# Autodesk Inventor assembly: roller-hand-v2-P
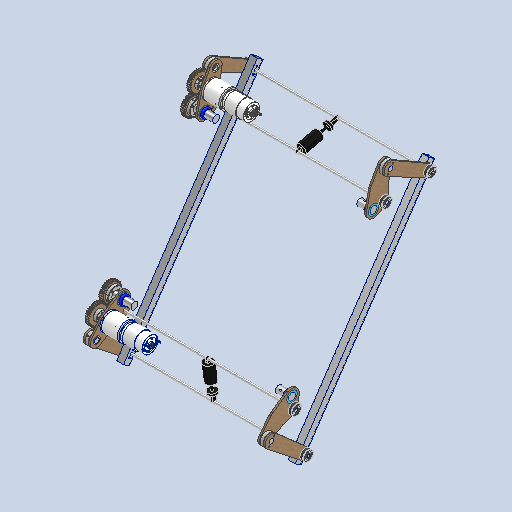
[picture p0: Inventor's stored thumbnail of the model, 512x512]
Saved by Autodesk Inventor 2025.1 (Build 291241000, 241)
## iProperties
Created: 2024-10-06
Part Number: roller-hand-v2-P
Document SubType Name: Assembly
Designer: haruy
Author: haruy
## Documents named in this file (38)
- C:\Users\haruy\Documents\ロボコン\NHK2025\cad\nagahisa\hand\roller\roller-hand-v2-P.iam
- C:\Users\haruy\Documents\ロボコン\NHK2025\cad\nagahisa\hand\roller\roller-hand-v1-MDF-m385-m.ipt
- C:\Users\haruy\Documents\ロボコン\NHK2025\cad\nagahisa\hand\roller\roller-hand-v2-MDF-link-1.ipt
- C:\Users\haruy\Documents\ロボコン\NHK2025\cad\nagahisa\hand\roller\roller-hand-v2-MDF-m385-r.ipt
- C:\Users\haruy\Documents\ロボコン\NHK2025\cad\nagahisa\hand\roller\SCSWJ8-6_b.ipt
- C:\Users\haruy\Documents\ロボコン\NHK2025\cad\000_parts\ベアリング\8\bear_f8_12_sa.ipt
- C:\Users\haruy\Documents\ロボコン\NHK2025\cad\000_parts\モーター\Geared_RS-385.iam
- C:\Users\haruy\Documents\ロボコン\NHK2025\cad\nagahisa\hand\roller\SCSWJ6-6_b.ipt
- C:\Users\haruy\Documents\ロボコン\NHK2025\cad\000_parts\ベアリング\12\TH22_bearing_12_18_19.5_sn.ipt
- C:\Users\haruy\Documents\ロボコン\NHK2025\cad\nagahisa\hand\roller\roller-hand-v2-Shaft-link1.ipt
- C:\Users\haruy\Documents\ロボコン\NHK2025\cad\nagahisa\hand\roller\roller-hand-v2-Shaft-link2.ipt
- C:\Users\haruy\Documents\ロボコン\NHK2025\cad\nagahisa\hand\roller\roller-hand-v2-Shaft-m.ipt
- C:\Users\haruy\Documents\ロボコン\NHK2025\cad\nagahisa\hand\roller\SCSWJ12-6_b.ipt
- C:\Users\haruy\Documents\ロボコン\NHK2025\cad\000_parts\サスペンション\black-suspension.iam
- C:\Users\haruy\Documents\ロボコン\NHK2025\cad\nagahisa\hand\roller\roller-hand-v2-Shaft-link3.ipt
- C:\Users\haruy\Documents\ロボコン\NHK2025\cad\nagahisa\hand\roller\roller-hand-v2-Shaft-m-r.ipt
- C:\Users\haruy\Documents\ロボコン\NHK2025\cad\nagahisa\hand\roller\roller-hand-v2-ASP-1.ipt
- C:\Users\haruy\Documents\ロボコン\NHK2025\cad\nagahisa\hand\roller\SCSWJ4-6_b.ipt
- C:\Users\haruy\Documents\ロボコン\NHK2025\cad\nagahisa\hand\roller\roller-hand-v2-P\デザイン アクセラレータ\平歯車1.iam
- C:\Users\haruy\Documents\ロボコン\NHK2025\cad\nagahisa\hand\roller\roller-hand-v2-3DP-shaft-spesa.ipt
- C:\Users\haruy\Documents\ロボコン\NHK2025\cad\nagahisa\hand\roller\roller-hand-v1-MDF-m385-m_MIR.ipt
- C:\Users\haruy\Documents\ロボコン\NHK2025\cad\nagahisa\hand\roller\roller-hand-v2-MDF-link-1_MIR.ipt
- C:\Users\haruy\Documents\ロボコン\NHK2025\cad\nagahisa\hand\roller\roller-hand-v2-MDF-m385-r_MIR.ipt
- C:\Users\haruy\Documents\ロボコン\NHK2025\cad\nagahisa\hand\roller\SCSWJ8-6_b_MIR.ipt
- C:\Users\haruy\Documents\ロボコン\NHK2025\cad\000_parts\モーター\Geared_RS-385_MIR.iam
- C:\Users\haruy\Documents\ロボコン\NHK2025\cad\nagahisa\hand\roller\SCSWJ6-6_b_MIR.ipt
- C:\Users\haruy\Documents\ロボコン\NHK2025\cad\000_parts\ベアリング\12\TH22_bearing_12_18_19.5_sn_MIR.ipt
- C:\Users\haruy\Documents\ロボコン\NHK2025\cad\nagahisa\hand\roller\roller-hand-v2-Shaft-link1_MIR.ipt
- C:\Users\haruy\Documents\ロボコン\NHK2025\cad\000_parts\ベアリング\8\bear_f8_12_sa_MIR.ipt
- C:\Users\haruy\Documents\ロボコン\NHK2025\cad\nagahisa\hand\roller\roller-hand-v2-Shaft-link2_MIR.ipt
- C:\Users\haruy\Documents\ロボコン\NHK2025\cad\nagahisa\hand\roller\roller-hand-v2-Shaft-m_MIR.ipt
- C:\Users\haruy\Documents\ロボコン\NHK2025\cad\nagahisa\hand\roller\SCSWJ12-6_b_MIR.ipt
- C:\Users\haruy\Documents\ロボコン\NHK2025\cad\000_parts\サスペンション\black-suspension_MIR.iam
- C:\Users\haruy\Documents\ロボコン\NHK2025\cad\nagahisa\hand\roller\roller-hand-v2-Shaft-link3_MIR.ipt
- C:\Users\haruy\Documents\ロボコン\NHK2025\cad\nagahisa\hand\roller\roller-hand-v2-Shaft-m-r_MIR.ipt
- C:\Users\haruy\Documents\ロボコン\NHK2025\cad\nagahisa\hand\roller\SCSWJ4-6_b_MIR.ipt
- C:\Users\haruy\Documents\ロボコン\NHK2025\cad\nagahisa\hand\roller\roller-hand-v2-P\デザイン アクセラレータ\平歯車1_MIR.iam
- C:\Users\haruy\Documents\ロボコン\NHK2025\cad\nagahisa\hand\roller\roller-hand-v2-3DP-shaft-spesa_MIR.ipt
## Components (55 placed, 37 different names)
1. roller-hand-v1-MDF-m385-m:1 — 挿入:4, 挿入:6, 挿入:8, 挿入:16, 挿入:21, 挿入:35
2. roller-hand-v2-MDF-link-1:1 — 挿入:7, 挿入:10, 挿入:22, 挿入:23, 挿入:27, 挿入:28, 挿入:34
3. roller-hand-v2-MDF-m385-r:1 — 挿入:12, 挿入:18, 挿入:25, 挿入:37
4. SCSWJ8-6_b:1 — 挿入:7, 挿入:9
5. bear_f8_12_sa:1 — 挿入:8, 挿入:9
6. Geared_RS-385:1 [sub-assembly] — 挿入:4, 挿入:5, メイト:1
7. SCSWJ6-6_b:1 — 挿入:5, メイト:2
8. TH22_bearing_12_18_19.5_sn:1 — 挿入:6, 挿入:19, 挿入:38, 挿入:39
9. roller-hand-v2-Shaft-link1:1 — 挿入:10, 挿入:29
10. TH22_bearing_12_18_19.5_sn:2 — 挿入:25, 挿入:26, 挿入:40
11. bear_f8_12_sa:2 — 挿入:12, 挿入:13
12. SCSWJ8-6_b:2 — 挿入:13, 挿入:31
13. roller-hand-v2-MDF-link-1:2 — 挿入:29, 挿入:30, 挿入:31, 挿入:32, 挿入:33, 挿入:36
14. roller-hand-v2-Shaft-link2:1 — 挿入:16, 挿入:18
15. roller-hand-v2-Shaft-m:1 — 挿入:19, メイト:3
16. SCSWJ12-6_b:1 — 挿入:38
17. black-suspension:1 [sub-assembly] — 挿入:21, 挿入:22
18. roller-hand-v2-Shaft-link3:1 — 挿入:23
19. roller-hand-v2-Shaft-link3:2 — 挿入:30
20. roller-hand-v2-Shaft-m-r:1 — 挿入:26
21. roller-hand-v2-ASP-1:1 — 挿入:27, 挿入:28, フラッシュ:1
22. roller-hand-v2-ASP-1:2 — 挿入:32, 挿入:33, 挿入:64, 挿入:65
23. SCSWJ4-6_b:1 — 挿入:35
24. SCSWJ4-6_b:2 — 挿入:34
25. SCSWJ4-6_b:3 — 挿入:36
26. SCSWJ4-6_b:4 — 挿入:37
27. 平歯車:1 [sub-assembly] — メイト:1, メイト:2, メイト:3
28. roller-hand-v2-3DP-shaft-spesa:1 — 挿入:39
29. roller-hand-v2-3DP-shaft-spesa:2 — 挿入:40
30. roller-hand-v1-MDF-m385-m_MIR:1 — 挿入:42, 挿入:44, 挿入:52, 挿入:56, 挿入:59, 挿入:66
31. roller-hand-v2-MDF-link-1_MIR:1 — 挿入:41, 挿入:45, 挿入:55, 挿入:60
32. roller-hand-v2-MDF-m385-r_MIR:1 — 挿入:46, 挿入:47, 挿入:51, 挿入:61
33. SCSWJ8-6_b_MIR:1 — 挿入:41, 挿入:67
34. Geared_RS-385_MIR:1 [sub-assembly] — 挿入:42, 挿入:43, メイト:6
35. SCSWJ6-6_b_MIR:1 — 挿入:43, メイト:5
36. TH22_bearing_12_18_19.5_sn_MIR:1 — 挿入:44, 挿入:53, 挿入:54, 挿入:62
37. roller-hand-v2-Shaft-link1_MIR:1 — 挿入:45, 挿入:50
38. TH22_bearing_12_18_19.5_sn_MIR:2 — 挿入:46, 挿入:58, 挿入:63
39. bear_f8_12_sa_MIR:1 — 挿入:47, 挿入:48
40. SCSWJ8-6_b_MIR:2 — 挿入:48, 挿入:49
41. roller-hand-v2-MDF-link-1_MIR:2 — 挿入:49, 挿入:50, 挿入:57, 挿入:64, 挿入:65, 挿入:68
42. roller-hand-v2-Shaft-link2_MIR:1 — 挿入:51, 挿入:52
43. roller-hand-v2-Shaft-m_MIR:1 — 挿入:53, メイト:4
44. SCSWJ12-6_b_MIR:1 — 挿入:54
45. black-suspension_MIR:1 [sub-assembly] — 挿入:55, 挿入:56
46. roller-hand-v2-Shaft-link3_MIR:1 — 挿入:57
47. roller-hand-v2-Shaft-m-r_MIR:1 — 挿入:58
48. SCSWJ4-6_b_MIR:1 — 挿入:59
49. SCSWJ4-6_b_MIR:2 — 挿入:60
50. SCSWJ4-6_b_MIR:3 — 挿入:61
51. 平歯車1_MIR:1 [sub-assembly] — メイト:4, メイト:5, メイト:6
52. roller-hand-v2-3DP-shaft-spesa_MIR:1 — 挿入:62
53. roller-hand-v2-3DP-shaft-spesa_MIR:2 — 挿入:63
54. bear_f8_12_sa:3 — 挿入:66, 挿入:67
55. SCSWJ4-6_b:5 — 挿入:68
## Relationships (66: Insert 59, Mate 6, Flush 1)
- 挿入:4 [Insert]: roller-hand-v1-MDF-m385-m:1 ↔ Geared_RS-385:1
- 挿入:5 [Insert] (8.8 mm): Geared_RS-385:1 ↔ SCSWJ6-6_b:1
- 挿入:6 [Insert]: roller-hand-v1-MDF-m385-m:1 ↔ TH22_bearing_12_18_19.5_sn:1
- 挿入:7 [Insert]: roller-hand-v2-MDF-link-1:1 ↔ SCSWJ8-6_b:1
- 挿入:8 [Insert]: roller-hand-v1-MDF-m385-m:1 ↔ bear_f8_12_sa:1
- 挿入:9 [Insert]: SCSWJ8-6_b:1 ↔ bear_f8_12_sa:1
- 挿入:10 [Insert] (-6.2 mm): roller-hand-v2-MDF-link-1:1 ↔ roller-hand-v2-Shaft-link1:1
- 挿入:12 [Insert]: roller-hand-v2-MDF-m385-r:1 ↔ bear_f8_12_sa:2
- 挿入:13 [Insert]: bear_f8_12_sa:2 ↔ SCSWJ8-6_b:2
- 挿入:16 [Insert] (-6 mm): roller-hand-v1-MDF-m385-m:1 ↔ roller-hand-v2-Shaft-link2:1
- 挿入:18 [Insert] (6 mm): roller-hand-v2-MDF-m385-r:1 ↔ roller-hand-v2-Shaft-link2:1
- 挿入:19 [Insert] (-18 mm): TH22_bearing_12_18_19.5_sn:1 ↔ roller-hand-v2-Shaft-m:1
- 挿入:21 [Insert] (143 mm): roller-hand-v1-MDF-m385-m:1 ↔ black-suspension:1
- 挿入:22 [Insert] (152.8 mm): roller-hand-v2-MDF-link-1:1 ↔ black-suspension:1
- 挿入:23 [Insert]: roller-hand-v2-MDF-link-1:1 ↔ roller-hand-v2-Shaft-link3:1
- 挿入:25 [Insert]: roller-hand-v2-MDF-m385-r:1 ↔ TH22_bearing_12_18_19.5_sn:2
- 挿入:26 [Insert]: TH22_bearing_12_18_19.5_sn:2 ↔ roller-hand-v2-Shaft-m-r:1
- 挿入:27 [Insert]: roller-hand-v2-MDF-link-1:1 ↔ roller-hand-v2-ASP-1:1
- 挿入:28 [Insert]: roller-hand-v2-MDF-link-1:1 ↔ roller-hand-v2-ASP-1:1
- 挿入:29 [Insert] (6.2 mm): roller-hand-v2-Shaft-link1:1 ↔ roller-hand-v2-MDF-link-1:2
- 挿入:30 [Insert]: roller-hand-v2-MDF-link-1:2 ↔ roller-hand-v2-Shaft-link3:2
- 挿入:31 [Insert]: SCSWJ8-6_b:2 ↔ roller-hand-v2-MDF-link-1:2
- 挿入:32 [Insert]: roller-hand-v2-MDF-link-1:2 ↔ roller-hand-v2-ASP-1:2
- 挿入:33 [Insert]: roller-hand-v2-MDF-link-1:2 ↔ roller-hand-v2-ASP-1:2
- 挿入:34 [Insert]: roller-hand-v2-MDF-link-1:1 ↔ SCSWJ4-6_b:2
- 挿入:35 [Insert]: roller-hand-v1-MDF-m385-m:1 ↔ SCSWJ4-6_b:1
- 挿入:36 [Insert]: roller-hand-v2-MDF-link-1:2 ↔ SCSWJ4-6_b:3
- 挿入:37 [Insert]: roller-hand-v2-MDF-m385-r:1 ↔ SCSWJ4-6_b:4
- メイト:1 [Mate]: Geared_RS-385:1 ↔ 平歯車:1
- メイト:2 [Mate]: SCSWJ6-6_b:1 ↔ 平歯車:1
- メイト:3 [Mate]: roller-hand-v2-Shaft-m:1 ↔ 平歯車:1
- 挿入:38 [Insert] (9.8 mm): TH22_bearing_12_18_19.5_sn:1 ↔ SCSWJ12-6_b:1
- 挿入:39 [Insert]: TH22_bearing_12_18_19.5_sn:1 ↔ roller-hand-v2-3DP-shaft-spesa:1
- 挿入:40 [Insert]: TH22_bearing_12_18_19.5_sn:2 ↔ roller-hand-v2-3DP-shaft-spesa:2
- フラッシュ:1 [Flush] (-206.5 mm): roller-hand-v2-ASP-1:1
- 挿入:41 [Insert]: roller-hand-v2-MDF-link-1_MIR:1 ↔ SCSWJ8-6_b_MIR:1
- 挿入:42 [Insert]: roller-hand-v1-MDF-m385-m_MIR:1 ↔ Geared_RS-385_MIR:1
- 挿入:43 [Insert] (8.8 mm): Geared_RS-385_MIR:1 ↔ SCSWJ6-6_b_MIR:1
- 挿入:44 [Insert]: roller-hand-v1-MDF-m385-m_MIR:1 ↔ TH22_bearing_12_18_19.5_sn_MIR:1
- 挿入:45 [Insert] (-6.2 mm): roller-hand-v2-MDF-link-1_MIR:1 ↔ roller-hand-v2-Shaft-link1_MIR:1
- 挿入:46 [Insert]: roller-hand-v2-MDF-m385-r_MIR:1 ↔ TH22_bearing_12_18_19.5_sn_MIR:2
- 挿入:47 [Insert]: roller-hand-v2-MDF-m385-r_MIR:1 ↔ bear_f8_12_sa_MIR:1
- 挿入:48 [Insert]: bear_f8_12_sa_MIR:1 ↔ SCSWJ8-6_b_MIR:2
- 挿入:49 [Insert]: SCSWJ8-6_b_MIR:2 ↔ roller-hand-v2-MDF-link-1_MIR:2
- 挿入:50 [Insert] (6.2 mm): roller-hand-v2-Shaft-link1_MIR:1 ↔ roller-hand-v2-MDF-link-1_MIR:2
- 挿入:51 [Insert] (6 mm): roller-hand-v2-MDF-m385-r_MIR:1 ↔ roller-hand-v2-Shaft-link2_MIR:1
- 挿入:52 [Insert] (-6 mm): roller-hand-v1-MDF-m385-m_MIR:1 ↔ roller-hand-v2-Shaft-link2_MIR:1
- 挿入:53 [Insert] (-18 mm): TH22_bearing_12_18_19.5_sn_MIR:1 ↔ roller-hand-v2-Shaft-m_MIR:1
- 挿入:54 [Insert] (9.8 mm): TH22_bearing_12_18_19.5_sn_MIR:1 ↔ SCSWJ12-6_b_MIR:1
- 挿入:55 [Insert] (152.8 mm): roller-hand-v2-MDF-link-1_MIR:1 ↔ black-suspension_MIR:1
- 挿入:56 [Insert] (143 mm): roller-hand-v1-MDF-m385-m_MIR:1 ↔ black-suspension_MIR:1
- 挿入:57 [Insert]: roller-hand-v2-MDF-link-1_MIR:2 ↔ roller-hand-v2-Shaft-link3_MIR:1
- 挿入:58 [Insert]: TH22_bearing_12_18_19.5_sn_MIR:2 ↔ roller-hand-v2-Shaft-m-r_MIR:1
- 挿入:59 [Insert]: roller-hand-v1-MDF-m385-m_MIR:1 ↔ SCSWJ4-6_b_MIR:1
- 挿入:60 [Insert]: roller-hand-v2-MDF-link-1_MIR:1 ↔ SCSWJ4-6_b_MIR:2
- 挿入:61 [Insert]: roller-hand-v2-MDF-m385-r_MIR:1 ↔ SCSWJ4-6_b_MIR:3
- メイト:4 [Mate]: roller-hand-v2-Shaft-m_MIR:1 ↔ 平歯車1_MIR:1
- メイト:5 [Mate]: SCSWJ6-6_b_MIR:1 ↔ 平歯車1_MIR:1
- メイト:6 [Mate]: Geared_RS-385_MIR:1 ↔ 平歯車1_MIR:1
- 挿入:62 [Insert]: TH22_bearing_12_18_19.5_sn_MIR:1 ↔ roller-hand-v2-3DP-shaft-spesa_MIR:1
- 挿入:63 [Insert]: TH22_bearing_12_18_19.5_sn_MIR:2 ↔ roller-hand-v2-3DP-shaft-spesa_MIR:2
- 挿入:64 [Insert]: roller-hand-v2-ASP-1:2 ↔ roller-hand-v2-MDF-link-1_MIR:2
- 挿入:65 [Insert]: roller-hand-v2-ASP-1:2 ↔ roller-hand-v2-MDF-link-1_MIR:2
- 挿入:66 [Insert]: roller-hand-v1-MDF-m385-m_MIR:1 ↔ bear_f8_12_sa:3
- 挿入:67 [Insert]: SCSWJ8-6_b_MIR:1 ↔ bear_f8_12_sa:3
- 挿入:68 [Insert]: roller-hand-v2-MDF-link-1_MIR:2 ↔ SCSWJ4-6_b:5
